# Autodesk Inventor assembly: ClawAssembly
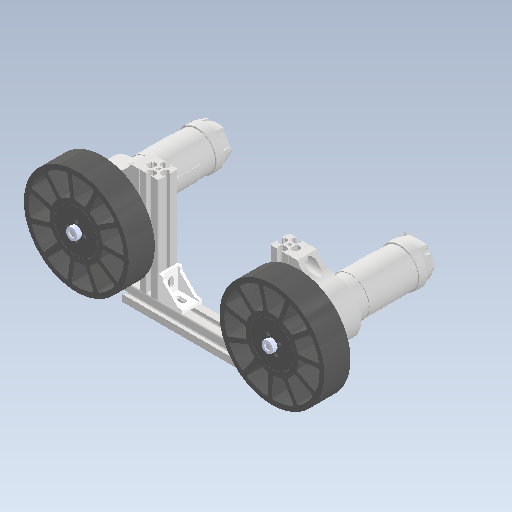
[picture p0: Inventor's stored thumbnail of the model, 512x512]
Saved by Autodesk Inventor 2020 (Build 240168000, 168)
## iProperties
Created: 2020-01-29
Part Number: ClawAssembly
Document SubType Name: Assembly
Designer: Jimmy
Author: Jimmy
## Documents named in this file (9)
- C:\Users\maple\Documents\GitHub\CAD\Robotics 2019-2020\Assembly\Pulley and Claw\Claw\ClawAssembly.iam
- C:\Users\maple\Documents\GitHub\CAD\Robotics 2019-2020\Assembly\Pulley and Claw\Claw\RevHexMotor\RevHexMotor.iam
- C:\Users\maple\Documents\GitHub\CAD\Robotics 2019-2020\Assembly\Pulley and Claw\Claw\AndymarkCompliantWheels\CompliantWheel.iam
- C:\Users\maple\Documents\GitHub\CAD\Robotics 2019-2020\Assembly\Pulley and Claw\Claw\MotorMount_vCAD.ipt
- C:\Users\maple\Documents\GitHub\CAD\Robotics 2019-2020\Assembly\Pulley and Claw\Claw\ShaftCollar.ipt
- C:\Users\maple\Documents\GitHub\CAD\Robotics 2019-2020\Assembly\Pulley and Claw\Claw\HexHub.ipt
- C:\Users\maple\Documents\GitHub\CAD\Robotics 2019-2020\Assembly\Pulley and Claw\Claw\Extrusions\4in.ipt
- C:\Users\maple\Documents\GitHub\CAD\Robotics 2019-2020\Assembly\Pulley and Claw\Claw\CornerBracket.ipt
- C:\Users\maple\Documents\GitHub\CAD\Robotics 2019-2020\Assembly\Pulley and Claw\Claw\Extrusions\7in.ipt
## Components (15 placed, 8 different names)
1. RevHexMotor:2 [sub-assembly] — Insert:3, Insert:4, Mate:1, Mate:2, Mate:3
2. CompliantWheel:1 [sub-assembly] — Insert:5, Insert:6, Insert:7
3. MotorMount_vCAD:1 — Insert:3, Insert:4, Mate:7, Flush:2, Flush:9
4. ShaftCollar:1 — Insert:7
5. HexHub:1 — Insert:5, Insert:6, Mate:1, Mate:2, Mate:3
6. RevHexMotor:3 [sub-assembly] — Insert:13, Insert:14
7. CompliantWheel:2 [sub-assembly]
8. MotorMount_vCAD:2 — Flush:3, Mate:8, Flush:4, Insert:13, Insert:14
9. ShaftCollar:2
10. HexHub:2
11. 4in:1 — Mate:7, Flush:2, Flush:9, Mate:11, Flush:14, Flush:16, Mate:12
12. 4in:2 — Flush:3, Mate:8, Flush:4, Flush:12, Flush:13, Mate:9
13. 7in:1 — Flush:10, Flush:11, Mate:10, Flush:15, Flush:17, Mate:12
14. CornerBracket:1 — Flush:10, Flush:11, Flush:12, Flush:13, Mate:9, Mate:10
15. CornerBracket:2 — Mate:11, Flush:14, Flush:15, Flush:16, Flush:17
## Relationships (34: Mate 12, Flush 12, Insert 10)
- Insert:3: RevHexMotor:2 ↔ MotorMount_vCAD:1
- Insert:4: RevHexMotor:2 ↔ MotorMount_vCAD:1
- Insert:5: CompliantWheel:1 ↔ HexHub:1
- Insert:6: CompliantWheel:1 ↔ HexHub:1
- Mate:1: RevHexMotor:2 ↔ HexHub:1
- Mate:2: RevHexMotor:2 ↔ HexHub:1
- Mate:3: RevHexMotor:2 ↔ HexHub:1
- Insert:7: CompliantWheel:1 ↔ ShaftCollar:1
- [Insert]: CompliantWheel:2 ↔ HexHub:2
- [Insert]: CompliantWheel:2 ↔ HexHub:2
- [Mate]: RevHexMotor:3 ↔ HexHub:2
- [Mate]: RevHexMotor:3 ↔ HexHub:2
- [Mate]: RevHexMotor:3 ↔ HexHub:2
- [Insert]: CompliantWheel:2 ↔ ShaftCollar:2
- Mate:7: MotorMount_vCAD:1 ↔ 4in:1
- Flush:2: MotorMount_vCAD:1 ↔ 4in:1
- Flush:3: MotorMount_vCAD:2 ↔ 4in:2
- Mate:8: MotorMount_vCAD:2 ↔ 4in:2
- Flush:4: MotorMount_vCAD:2 ↔ 4in:2
- Insert:13: RevHexMotor:3 ↔ MotorMount_vCAD:2
- Insert:14: RevHexMotor:3 ↔ MotorMount_vCAD:2
- Flush:9: MotorMount_vCAD:1 ↔ 4in:1
- Flush:10: 7in:1 ↔ CornerBracket:1
- Flush:11 (34.925 mm): 7in:1 ↔ CornerBracket:1
- Flush:12: 4in:2 ↔ CornerBracket:1
- Flush:13: 4in:2 ↔ CornerBracket:1
- Mate:9: 4in:2 ↔ CornerBracket:1
- Mate:10: 7in:1 ↔ CornerBracket:1
- Mate:11: 4in:1 ↔ CornerBracket:2
- Flush:14: 4in:1 ↔ CornerBracket:2
- Flush:15: 7in:1 ↔ CornerBracket:2
- Flush:16: 4in:1 ↔ CornerBracket:2
- Flush:17 (34.925 mm): 7in:1 ↔ CornerBracket:2
- Mate:12: 4in:1 ↔ 7in:1
## Named parameters: d43_d37 = 0 mm, d44_d38 = 0 mm, d45_d39 = 0 mm, d46_d40 = 0 mm, d47_d42 = 0 mm, d50_d36 = 0 mm
